# Autodesk Inventor assembly: simple_plate_assembly_stacked
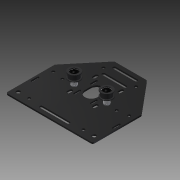
[picture p0: Inventor's stored thumbnail of the model, 180x180]
Saved by Autodesk Inventor 2014 (Build 180170000, 170)
## iProperties
Created: 2013-05-29
Part Number: simple_plate_assembly_stacked
Document SubType Name: Assembly
Designer: Edward
Mass: 864.739 g
Surface Area: 894.967 cm^2
Volume: 163.574 cm^3
Density: 5.28654 g/cm^3
Author: Edward
## Documents named in this file (7)
- C:\Users\Edward\Documents\Vault\Designs\Shapeoko_v2\v2_final\simple_plate_assembly_stacked.iam
- C:\Users\Edward\Documents\Vault\Designs\Shapeoko_v2\v2_final\26029-01.ipt
- C:\Users\Edward\Documents\Vault\Designs\Shapeoko_v2\v2_final\25287-02.ipt
- C:\Users\Edward\Documents\Vault\Designs\Shapeoko_v2\v2_final\25284-02.ipt
- C:\Users\Edward\Documents\Vault\Designs\Shapeoko_v2\v2_final\25197-02.iam
- C:\Users\Edward\Documents\Vault\Designs\Shapeoko_v2\v2_final\25286-05.ipt
- C:\Users\Edward\Documents\Vault\Designs\Shapeoko_v2\v2_final\25312-14.ipt
## Components (15 placed, 6 different names)
1. 26029-01:1 — Insert:21, Insert:24, Insert:26, Insert:43
2. 25197-02:1 [sub-assembly]
3. 25197-02:2 [sub-assembly] — Insert:21
4. 25286-05:2
5. 25287-02:8 — Insert:23, Insert:24
6. 25284-02:4 — Insert:23
7. 25286-05:1
8. 25284-02:5 — Insert:27
9. 25287-02:9 — Insert:26, Insert:27
10. 25312-14:1 — Insert:40
11. 25312-14:2 — Insert:42
12. 25287-02:10 — Insert:39
13. 25287-02:11 — Insert:39, Insert:40
14. 25287-02:12 — Insert:41, Insert:43
15. 25287-02:13 — Insert:41, Insert:42
## Relationships (14: Insert 14)
- Insert:21 (9.525 mm): 26029-01:1 ↔ 25197-02:2
- [Insert]: 25197-02:1 ↔ 25286-05:2
- Insert:23: 25287-02:8 ↔ 25284-02:4
- Insert:24: 26029-01:1 ↔ 25287-02:8
- [Insert]: 25197-02:2 ↔ 25286-05:1
- Insert:26: 26029-01:1 ↔ 25287-02:9
- Insert:27: 25284-02:5 ↔ 25287-02:9
- [Insert]: 25197-02:2 ↔ 25312-14:1
- [Insert]: 25197-02:1 ↔ 25312-14:2
- Insert:39: 25287-02:10 ↔ 25287-02:11
- Insert:40: 25312-14:1 ↔ 25287-02:11
- Insert:41: 25287-02:12 ↔ 25287-02:13
- Insert:42: 25312-14:2 ↔ 25287-02:13
- Insert:43: 26029-01:1 ↔ 25287-02:12
